# Autodesk Inventor assembly: Neo550Assembly
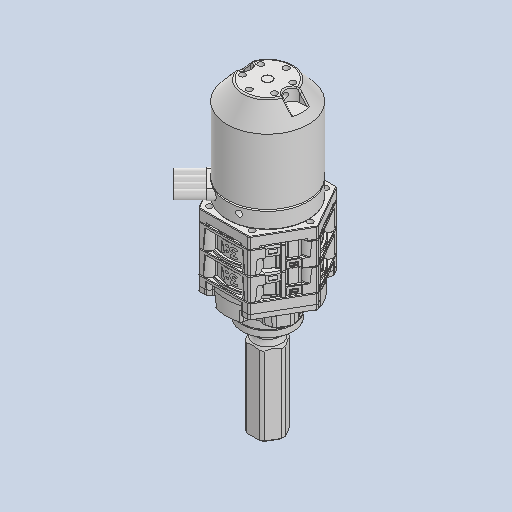
[picture p0: Inventor's stored thumbnail of the model, 512x512]
Saved by Autodesk Inventor 2022 (Build 260153000, 153)
## iProperties
Created: 2022-01-17
Part Number: Neo550Assembly
Document SubType Name: Assembly
Designer: Ty Gazaway
Author: Ty Gazaway
## Documents named in this file (6)
- C:\Users\tagaz\OneDrive\Documents\T3-Cad\CAD\Generic and Stock\RevMotorParts\Neo550Assembly.iam
- C:\Users\tagaz\OneDrive\Documents\T3-Cad\CAD\Generic and Stock\Neo550.ipt
- C:\Users\tagaz\OneDrive\Documents\T3-Cad\CAD\Generic and Stock\RevMotorParts\UltraPlan3_1Stage.ipt
- C:\Users\tagaz\OneDrive\Documents\T3-Cad\CAD\Generic and Stock\RevMotorParts\FemaleConnector.ipt
- C:\Users\tagaz\OneDrive\Documents\T3-Cad\CAD\Generic and Stock\RevMotorParts\HexShaftConvert.ipt
- C:\Users\tagaz\OneDrive\Documents\T3-Cad\CAD\Generic and Stock\RevMotorParts\ultraPlate.ipt
## Components (6 placed, 5 different names)
1. Neo550:1 — Mate:1, Insert:1
2. UltraPlan3_1Stage:1 — Mate:3, Mate:4, Mate:5, Mate:6, Mate:7
3. UltraPlan3_1Stage:2 — Mate:6, Mate:7, Mate:8, Mate:9, Mate:10, Mate:11
4. FemaleConnector:1 — Mate:9, Mate:10, Mate:11, Mate:12, Insert:2
5. HexShaftConvert:1 — Mate:12, Insert:2
6. ultraPlate:1 — Mate:1, Insert:1, Mate:3, Mate:4, Mate:5, Mate:8
## Relationships (13: Mate 11, Insert 2)
- Mate:1: Neo550:1 ↔ ultraPlate:1
- Insert:1: Neo550:1 ↔ ultraPlate:1
- Mate:3: UltraPlan3_1Stage:1 ↔ ultraPlate:1
- Mate:4: UltraPlan3_1Stage:1 ↔ ultraPlate:1
- Mate:5: UltraPlan3_1Stage:1 ↔ ultraPlate:1
- Mate:6: UltraPlan3_1Stage:1 ↔ UltraPlan3_1Stage:2
- Mate:7: UltraPlan3_1Stage:1 ↔ UltraPlan3_1Stage:2
- Mate:8: UltraPlan3_1Stage:2 ↔ ultraPlate:1
- Mate:9: UltraPlan3_1Stage:2 ↔ FemaleConnector:1
- Mate:10: UltraPlan3_1Stage:2 ↔ FemaleConnector:1
- Mate:11: UltraPlan3_1Stage:2 ↔ FemaleConnector:1
- Mate:12: FemaleConnector:1 ↔ HexShaftConvert:1
- Insert:2: FemaleConnector:1 ↔ HexShaftConvert:1
